# Autodesk Inventor assembly: ASY 9610 charging hatch
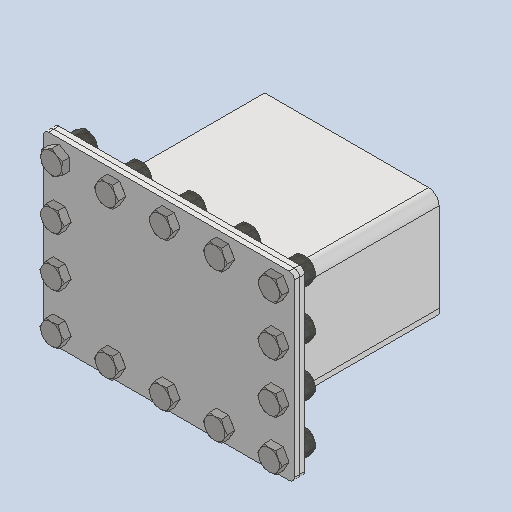
[picture p0: Inventor's stored thumbnail of the model, 512x512]
Saved by Autodesk Inventor 2026.2 (Build 302298000, 298)
## iProperties
Created: 2026-06-14
Part Number: ASY 9610 charging hatch
Document SubType Name: Assembly
Designer: admin
Author: admin
## Documents named in this file (7)
- C:\Users\admin\Documents\Inventor\PRS-Purovsk\ASY 9610 charging hatch.iam
- C:\Users\admin\Documents\Inventor\PRS-Purovsk\PRS 9607 charging flange rect_D1200.ipt
- C:\Users\admin\Documents\Inventor\PRS-Purovsk\PRS 9606 charging flange round_D1200.ipt
- C:\Users\admin\Documents\Inventor\PRS-Purovsk\PRS 9672 charging tube 2_D1200.ipt
- C:\Users\admin\Documents\Inventor\PRS-Purovsk\cc\en-US\ISO 4017(1)\ISO 4017 - M16 x 35 - ISO.ipt
- C:\Users\admin\Documents\Inventor\PRS-Purovsk\cc\en-US\ISO 7090\ISO 7090 - 16 - 140 HV(1).ipt
- C:\Users\admin\Documents\Inventor\PRS-Purovsk\cc\en-US\ISO 4033(2)\ISO 4033 - M16 - ISO.ipt
## Components (46 placed, 6 different names)
1. PRS 9607 charging flange rect_D1200:1 — Mate:59
2. PRS 9606 charging flange round_D1200:1
3. PRS 9672 charging tube 2_D1200:1 — Mate:57, Mate:58
4. PRS 9672 charging tube 2_D1200:2
5. ISO 4017 M16 x 35:1
6. ISO 7090 16 - 140 HV:1
7. ISO 4033 M16:1
8. ISO 4017 M16 x 35:2
9. ISO 4017 M16 x 35:3
10. ISO 4017 M16 x 35:4
11. ISO 4017 M16 x 35:5
12. ISO 4017 M16 x 35:6
13. ISO 4017 M16 x 35:7
14. ISO 4017 M16 x 35:8
15. ISO 4017 M16 x 35:9
16. ISO 4017 M16 x 35:10
17. ISO 4017 M16 x 35:11
18. ISO 4017 M16 x 35:12
19. ISO 4017 M16 x 35:13
20. ISO 4017 M16 x 35:14
21. ISO 7090 16 - 140 HV:2
22. ISO 7090 16 - 140 HV:3
23. ISO 7090 16 - 140 HV:4
24. ISO 7090 16 - 140 HV:5
25. ISO 7090 16 - 140 HV:6
26. ISO 7090 16 - 140 HV:7
27. ISO 7090 16 - 140 HV:8
28. ISO 7090 16 - 140 HV:9
29. ISO 7090 16 - 140 HV:10
30. ISO 7090 16 - 140 HV:11
31. ISO 7090 16 - 140 HV:12
32. ISO 7090 16 - 140 HV:13
33. ISO 7090 16 - 140 HV:14
34. ISO 4033 M16:2
35. ISO 4033 M16:3
36. ISO 4033 M16:4
37. ISO 4033 M16:5
38. ISO 4033 M16:6
39. ISO 4033 M16:7
40. ISO 4033 M16:8
41. ISO 4033 M16:9
42. ISO 4033 M16:10
43. ISO 4033 M16:11
44. ISO 4033 M16:12
45. ISO 4033 M16:13
46. ISO 4033 M16:14
## Relationships (76: Mate 59, Insert 14, WeldJoint 3)
- [WeldJoint]: PRS 9607 charging flange rect_D1200:1 ↔ PRS 9606 charging flange round_D1200:1
- [WeldJoint]: PRS 9672 charging tube 2_D1200:1 ↔ PRS 9672 charging tube 2_D1200:2
- [WeldJoint]: PRS 9606 charging flange round_D1200:1 ↔ PRS 9672 charging tube 2_D1200:2
- [Mate]: PRS 9607 charging flange rect_D1200:1 ↔ ISO 4017 M16 x 35:1
- [Mate]: PRS 9607 charging flange rect_D1200:1 ↔ ISO 4017 M16 x 35:1
- [Mate]: PRS 9607 charging flange rect_D1200:1 ↔ ISO 4017 M16 x 35:2
- [Mate]: PRS 9607 charging flange rect_D1200:1 ↔ ISO 4017 M16 x 35:2
- [Mate]: PRS 9607 charging flange rect_D1200:1 ↔ ISO 4017 M16 x 35:3
- [Mate]: PRS 9607 charging flange rect_D1200:1 ↔ ISO 4017 M16 x 35:3
- [Mate]: PRS 9607 charging flange rect_D1200:1 ↔ ISO 4017 M16 x 35:4
- [Mate]: PRS 9607 charging flange rect_D1200:1 ↔ ISO 4017 M16 x 35:4
- [Mate]: PRS 9607 charging flange rect_D1200:1 ↔ ISO 4017 M16 x 35:5
- [Mate]: PRS 9607 charging flange rect_D1200:1 ↔ ISO 4017 M16 x 35:5
- [Mate]: PRS 9607 charging flange rect_D1200:1 ↔ ISO 4017 M16 x 35:6
- [Mate]: PRS 9607 charging flange rect_D1200:1 ↔ ISO 4017 M16 x 35:6
- [Mate]: PRS 9607 charging flange rect_D1200:1 ↔ ISO 4017 M16 x 35:7
- [Mate]: PRS 9607 charging flange rect_D1200:1 ↔ ISO 4017 M16 x 35:7
- [Mate]: PRS 9607 charging flange rect_D1200:1 ↔ ISO 4017 M16 x 35:8
- [Mate]: PRS 9607 charging flange rect_D1200:1 ↔ ISO 4017 M16 x 35:8
- [Mate]: PRS 9607 charging flange rect_D1200:1 ↔ ISO 4017 M16 x 35:9
- [Mate]: PRS 9607 charging flange rect_D1200:1 ↔ ISO 4017 M16 x 35:9
- [Mate]: PRS 9607 charging flange rect_D1200:1 ↔ ISO 4017 M16 x 35:10
- [Mate]: PRS 9607 charging flange rect_D1200:1 ↔ ISO 4017 M16 x 35:10
- [Mate]: PRS 9607 charging flange rect_D1200:1 ↔ ISO 4017 M16 x 35:11
- [Mate]: PRS 9607 charging flange rect_D1200:1 ↔ ISO 4017 M16 x 35:11
- [Mate]: PRS 9607 charging flange rect_D1200:1 ↔ ISO 4017 M16 x 35:12
- [Mate]: PRS 9607 charging flange rect_D1200:1 ↔ ISO 4017 M16 x 35:12
- [Mate]: PRS 9607 charging flange rect_D1200:1 ↔ ISO 4017 M16 x 35:13
- [Mate]: PRS 9607 charging flange rect_D1200:1 ↔ ISO 4017 M16 x 35:13
- [Mate]: PRS 9607 charging flange rect_D1200:1 ↔ ISO 4017 M16 x 35:14
- [Mate]: PRS 9607 charging flange rect_D1200:1 ↔ ISO 4017 M16 x 35:14
- [Mate]: PRS 9607 charging flange rect_D1200:1 ↔ ISO 7090 16 - 140 HV:1
- [Mate]: PRS 9606 charging flange round_D1200:1 ↔ ISO 7090 16 - 140 HV:1
- [Mate]: PRS 9607 charging flange rect_D1200:1 ↔ ISO 7090 16 - 140 HV:2
- [Mate]: PRS 9606 charging flange round_D1200:1 ↔ ISO 7090 16 - 140 HV:2
- [Mate]: PRS 9607 charging flange rect_D1200:1 ↔ ISO 7090 16 - 140 HV:3
- [Mate]: PRS 9606 charging flange round_D1200:1 ↔ ISO 7090 16 - 140 HV:3
- [Mate]: PRS 9607 charging flange rect_D1200:1 ↔ ISO 7090 16 - 140 HV:4
- [Mate]: PRS 9606 charging flange round_D1200:1 ↔ ISO 7090 16 - 140 HV:4
- [Mate]: PRS 9607 charging flange rect_D1200:1 ↔ ISO 7090 16 - 140 HV:5
- [Mate]: PRS 9606 charging flange round_D1200:1 ↔ ISO 7090 16 - 140 HV:5
- [Mate]: PRS 9607 charging flange rect_D1200:1 ↔ ISO 7090 16 - 140 HV:6
- [Mate]: PRS 9606 charging flange round_D1200:1 ↔ ISO 7090 16 - 140 HV:6
- [Mate]: PRS 9607 charging flange rect_D1200:1 ↔ ISO 7090 16 - 140 HV:7
- [Mate]: PRS 9606 charging flange round_D1200:1 ↔ ISO 7090 16 - 140 HV:7
- [Mate]: PRS 9607 charging flange rect_D1200:1 ↔ ISO 7090 16 - 140 HV:8
- [Mate]: PRS 9606 charging flange round_D1200:1 ↔ ISO 7090 16 - 140 HV:8
- [Mate]: PRS 9607 charging flange rect_D1200:1 ↔ ISO 7090 16 - 140 HV:9
- [Mate]: PRS 9606 charging flange round_D1200:1 ↔ ISO 7090 16 - 140 HV:9
- [Mate]: PRS 9607 charging flange rect_D1200:1 ↔ ISO 7090 16 - 140 HV:10
- [Mate]: PRS 9606 charging flange round_D1200:1 ↔ ISO 7090 16 - 140 HV:10
- [Mate]: PRS 9607 charging flange rect_D1200:1 ↔ ISO 7090 16 - 140 HV:11
- [Mate]: PRS 9606 charging flange round_D1200:1 ↔ ISO 7090 16 - 140 HV:11
- [Mate]: PRS 9607 charging flange rect_D1200:1 ↔ ISO 7090 16 - 140 HV:12
- [Mate]: PRS 9606 charging flange round_D1200:1 ↔ ISO 7090 16 - 140 HV:12
- [Mate]: PRS 9607 charging flange rect_D1200:1 ↔ ISO 7090 16 - 140 HV:13
- [Mate]: PRS 9606 charging flange round_D1200:1 ↔ ISO 7090 16 - 140 HV:13
- [Mate]: PRS 9607 charging flange rect_D1200:1 ↔ ISO 7090 16 - 140 HV:14
- [Mate]: PRS 9606 charging flange round_D1200:1 ↔ ISO 7090 16 - 140 HV:14
- [Insert]: ISO 7090 16 - 140 HV:1 ↔ ISO 4033 M16:1
- [Insert]: ISO 7090 16 - 140 HV:2 ↔ ISO 4033 M16:2
- [Insert]: ISO 7090 16 - 140 HV:3 ↔ ISO 4033 M16:3
- [Insert]: ISO 7090 16 - 140 HV:4 ↔ ISO 4033 M16:4
- [Insert]: ISO 7090 16 - 140 HV:5 ↔ ISO 4033 M16:5
- [Insert]: ISO 7090 16 - 140 HV:6 ↔ ISO 4033 M16:6
- [Insert]: ISO 7090 16 - 140 HV:7 ↔ ISO 4033 M16:7
- [Insert]: ISO 7090 16 - 140 HV:8 ↔ ISO 4033 M16:8
- [Insert]: ISO 7090 16 - 140 HV:9 ↔ ISO 4033 M16:9
- [Insert]: ISO 7090 16 - 140 HV:10 ↔ ISO 4033 M16:10
- [Insert]: ISO 7090 16 - 140 HV:11 ↔ ISO 4033 M16:11
- [Insert]: ISO 7090 16 - 140 HV:12 ↔ ISO 4033 M16:12
- [Insert]: ISO 7090 16 - 140 HV:13 ↔ ISO 4033 M16:13
- [Insert]: ISO 7090 16 - 140 HV:14 ↔ ISO 4033 M16:14
- Mate:57: PRS 9672 charging tube 2_D1200:1
- Mate:58: PRS 9672 charging tube 2_D1200:1
- Mate:59: PRS 9607 charging flange rect_D1200:1
## Named parameters: d0_d67 = 0 mm, d1_d30 = 0 mm, d2_d72 = 0 mm
